# Autodesk Inventor assembly: yagi_Front
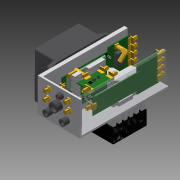
[picture p0: Inventor's stored thumbnail of the model, 180x180]
Saved by Autodesk Inventor 2014 (Build 180170000, 170)
## iProperties
Created: 2015-01-07
Part Number: yagi_Front
Document SubType Name: Assembly
Designer: Owner
Author: Owner
## Documents named in this file (22)
- C:\Users\Owner\Documents\APC\FrontEnd\IAM\Yagi\yagi_Front.iam
- C:\Users\Owner\Documents\APC\FrontEnd\IAM\Yagi\YagiBoard.iam
- C:\Users\Owner\Documents\APC\FrontEnd\IAM\Common\Yagi_BaseFrame.ipt
- C:\Users\Owner\Documents\APC\FrontEnd\IAM\Yagi\Yagi_Front_BackPlate.ipt
- C:\Users\Owner\Documents\APC\FrontEnd\IAM\Common\LED_Inset.ipt
- C:\Users\Owner\Documents\APC\FrontEnd\IAM\Common\BiglConnector.ipt
- C:\Users\Owner\Documents\APC\FrontEnd\IAM\Common\SmallConnector.ipt
- C:\Users\Owner\Documents\APC\FrontEnd\IAM\Yagi\SMA_Bulkhead.ipt
- C:\Users\Owner\Documents\APC\FrontEnd\IAM\Common\InjectorBoard2.iam
- C:\Users\Owner\Documents\APC\FrontEnd\IAM\Common\Peltier.ipt
- C:\Users\Owner\Documents\APC\FrontEnd\IAM\Common\PeltierPower.iam
- C:\Users\Owner\Documents\APC\FrontEnd\IAM\Common\Fan60.ipt
- C:\Users\Owner\Documents\APC\FrontEnd\IAM\Common\HeatSink60.ipt
- C:\Users\Owner\Documents\APC\FrontEnd\IAM\Common\NEAMBox.ipt
- C:\Users\Owner\Documents\APC\FrontEnd\IAM\Yagi\ColdFingerBase.ipt
- C:\Users\Owner\Documents\APC\FrontEnd\IAM\Yagi\ColdFingerStem.ipt
- C:\Users\Owner\Documents\APC\FrontEnd\IAM\Yagi\PeltierThermalSpacer.ipt
- C:\Users\Owner\Documents\APC\FrontEnd\IAM\Yagi\PeltierHeatSinkMount.ipt
- C:\Users\Owner\Documents\APC\FrontEnd\IAM\Yagi\YagiTop.ipt
- C:\Users\Owner\Documents\APC\FrontEnd\IAM\Common\PeltierController.iam
- C:\Users\Owner\Documents\APC\FrontEnd\IAM\Yagi\CavitySplitter.ipt
- C:\Users\Owner\Documents\APC\FrontEnd\IAM\Common\AmpPS.iam
## Components (27 placed, 21 different names)
1. YagiBoard:1 [sub-assembly] — Mate:47, Flush:16, Flush:17, Flush:48
2. Yagi_BaseFrame:1 — Flush:11, Mate:38, Flush:15, Mate:48, Flush:18, Flush:19, Flush:20, Flush:21, Mate:54, Flush:27, Flush:43, Flush:46, Mate:62
3. Yagi_BaseFrame:2 — Mate:47, Flush:16, Flush:17, Flush:20, Flush:21, Flush:22
4. Yagi_Front_BackPlate:1 — Mate:22, Mate:25, Mate:26, Mate:27, Mate:28, Mate:29, Mate:30, Mate:31, Flush:11, Mate:38, Flush:15, Mate:39, Mate:40, Mate:41, Mate:42, Mate:43, Mate:44, Mate:45, Mate:46, Angle:2, Angle:3, Angle:4, Angle:5, Flush:22, Flush:41, Flush:42
5. LED_Inset:2 — Mate:22, Mate:25
6. BiglConnector:1 — Mate:26, Mate:31
7. SmallConnector:1 — Mate:27, Mate:30
8. SmallConnector:2 — Mate:28, Mate:29
9. SMA_Bulkhead:1 — Mate:40, Mate:45, Angle:3
10. SMA_Bulkhead:2 — Mate:39, Mate:46, Angle:2
11. SMA_Bulkhead:3 — Mate:41, Mate:44, Angle:4
12. SMA_Bulkhead:4 — Mate:42, Mate:43, Angle:5
13. YagiBoard:2 [sub-assembly] — Mate:48, Flush:18, Flush:19
14. InjectorBoard2:1 [sub-assembly] — Mate:63, Flush:48, Mate:65, Flush:50
15. Peltier:1 — Flush:28, Flush:29, Flush:30, Flush:33, Flush:34, Flush:35
16. PeltierPower:1 [sub-assembly] — Mate:51, Mate:52, Mate:53
17. Fan60:1 — Mate:49, Flush:23, Flush:24, Flush:39, Flush:40, Flush:37, Flush:36
18. HeatSink60:1 — Mate:49, Flush:23, Flush:24, Mate:56, Flush:38
19. NEAMBox:1 — Mate:51, Mate:52, Mate:53, Mate:54, Flush:27, Mate:59, Mate:60, Flush:46
20. ColdFingerBase:1 — Flush:28, Flush:29, Flush:30, Mate:55, Flush:31, Mate:58
21. ColdFingerStem:1 — Mate:55, Flush:31, Mate:58
22. PeltierThermalSpacer:1 — Flush:33, Flush:34, Flush:35, Mate:56, Flush:36, Flush:37
23. PeltierHeatSinkMount:1 — Flush:38, Flush:39, Flush:40, Mate:57, Flush:44, Flush:45
24. YagiTop:1 — Flush:41, Flush:42, Flush:43, Mate:57, Flush:44, Flush:45, Mate:61, Flush:47
25. PeltierController:1 [sub-assembly] — Mate:59, Mate:60
26. CavitySplitter:1 — Mate:61, Mate:62, Mate:63, Flush:47, Mate:64, Flush:49, Flush:50
27. AmpPS:1 [sub-assembly] — Mate:64, Flush:49, Mate:65
## Relationships (73: Mate 35, Flush 34, Angle 4)
- Mate:22: Yagi_Front_BackPlate:1 ↔ LED_Inset:2
- Mate:25: Yagi_Front_BackPlate:1 ↔ LED_Inset:2
- Mate:26: Yagi_Front_BackPlate:1 ↔ BiglConnector:1
- Mate:27: Yagi_Front_BackPlate:1 ↔ SmallConnector:1
- Mate:28: Yagi_Front_BackPlate:1 ↔ SmallConnector:2
- Mate:29: Yagi_Front_BackPlate:1 ↔ SmallConnector:2
- Mate:30: Yagi_Front_BackPlate:1 ↔ SmallConnector:1
- Mate:31: Yagi_Front_BackPlate:1 ↔ BiglConnector:1
- Flush:11: Yagi_BaseFrame:1 ↔ Yagi_Front_BackPlate:1
- Mate:38: Yagi_BaseFrame:1 ↔ Yagi_Front_BackPlate:1
- Flush:15: Yagi_BaseFrame:1 ↔ Yagi_Front_BackPlate:1
- Mate:39: Yagi_Front_BackPlate:1 ↔ SMA_Bulkhead:2
- Mate:40: Yagi_Front_BackPlate:1 ↔ SMA_Bulkhead:1
- Mate:41: Yagi_Front_BackPlate:1 ↔ SMA_Bulkhead:3
- Mate:42: Yagi_Front_BackPlate:1 ↔ SMA_Bulkhead:4
- Mate:43: Yagi_Front_BackPlate:1 ↔ SMA_Bulkhead:4
- Mate:44: Yagi_Front_BackPlate:1 ↔ SMA_Bulkhead:3
- Mate:45: Yagi_Front_BackPlate:1 ↔ SMA_Bulkhead:1
- Mate:46: Yagi_Front_BackPlate:1 ↔ SMA_Bulkhead:2
- Angle:2 (0 deg): Yagi_Front_BackPlate:1 ↔ SMA_Bulkhead:2
- Angle:3 (0 deg): Yagi_Front_BackPlate:1 ↔ SMA_Bulkhead:1
- Angle:4 (0 deg): Yagi_Front_BackPlate:1 ↔ SMA_Bulkhead:3
- Angle:5 (0 deg): Yagi_Front_BackPlate:1 ↔ SMA_Bulkhead:4
- Mate:47 (3.175 mm): YagiBoard:1 ↔ Yagi_BaseFrame:2
- Flush:16: YagiBoard:1 ↔ Yagi_BaseFrame:2
- Flush:17 (3.175 mm): YagiBoard:1 ↔ Yagi_BaseFrame:2
- Mate:48 (3.175 mm): Yagi_BaseFrame:1 ↔ YagiBoard:2
- Flush:18 (3.175 mm): Yagi_BaseFrame:1 ↔ YagiBoard:2
- Flush:19: Yagi_BaseFrame:1 ↔ YagiBoard:2
- Flush:20: Yagi_BaseFrame:1 ↔ Yagi_BaseFrame:2
- Flush:21: Yagi_BaseFrame:1 ↔ Yagi_BaseFrame:2
- Flush:22: Yagi_BaseFrame:2 ↔ Yagi_Front_BackPlate:1
- Mate:49: Fan60:1 ↔ HeatSink60:1
- Flush:23 (-1 mm): Fan60:1 ↔ HeatSink60:1
- Flush:24 (-2 mm): Fan60:1 ↔ HeatSink60:1
- Mate:51: PeltierPower:1 ↔ NEAMBox:1
- Mate:52 (6.35 mm): PeltierPower:1 ↔ NEAMBox:1
- Mate:53 (3.175 mm): PeltierPower:1 ↔ NEAMBox:1
- Mate:54: Yagi_BaseFrame:1 ↔ NEAMBox:1
- Flush:27 (-3.175 mm): Yagi_BaseFrame:1 ↔ NEAMBox:1
- Flush:28: Peltier:1 ↔ ColdFingerBase:1
- Flush:29: Peltier:1 ↔ ColdFingerBase:1
- Flush:30: Peltier:1 ↔ ColdFingerBase:1
- Mate:55: ColdFingerBase:1 ↔ ColdFingerStem:1
- Flush:31: ColdFingerBase:1 ↔ ColdFingerStem:1
- Mate:58: ColdFingerBase:1 ↔ ColdFingerStem:1
- Flush:33: Peltier:1 ↔ PeltierThermalSpacer:1
- Flush:34: Peltier:1 ↔ PeltierThermalSpacer:1
- Flush:35: Peltier:1 ↔ PeltierThermalSpacer:1
- Mate:56: HeatSink60:1 ↔ PeltierThermalSpacer:1
- Flush:36 (10 mm): Fan60:1 ↔ PeltierThermalSpacer:1
- Flush:37 (10 mm): Fan60:1 ↔ PeltierThermalSpacer:1
- Flush:38: HeatSink60:1 ↔ PeltierHeatSinkMount:1
- Flush:39: Fan60:1 ↔ PeltierHeatSinkMount:1
- Flush:40: Fan60:1 ↔ PeltierHeatSinkMount:1
- Flush:41: Yagi_Front_BackPlate:1 ↔ YagiTop:1
- Flush:42: Yagi_Front_BackPlate:1 ↔ YagiTop:1
- Flush:43: Yagi_BaseFrame:1 ↔ YagiTop:1
- Mate:57: PeltierHeatSinkMount:1 ↔ YagiTop:1
- Flush:44: PeltierHeatSinkMount:1 ↔ YagiTop:1
- Flush:45: PeltierHeatSinkMount:1 ↔ YagiTop:1
- Mate:59: NEAMBox:1 ↔ PeltierController:1
- Mate:60 (6.35 mm): NEAMBox:1 ↔ PeltierController:1
- Flush:46 (38.1 mm): Yagi_BaseFrame:1 ↔ NEAMBox:1
- Mate:61: YagiTop:1 ↔ CavitySplitter:1
- Mate:62 (22.86 mm): Yagi_BaseFrame:1 ↔ CavitySplitter:1
- Mate:63: InjectorBoard2:1 ↔ CavitySplitter:1
- Flush:47: YagiTop:1 ↔ CavitySplitter:1
- Flush:48: YagiBoard:1 ↔ InjectorBoard2:1
- Mate:64 (1.5875 mm): CavitySplitter:1 ↔ AmpPS:1
- Flush:49: CavitySplitter:1 ↔ AmpPS:1
- Mate:65 (1.5875 mm): InjectorBoard2:1 ↔ AmpPS:1
- Flush:50 (3.175 mm): InjectorBoard2:1 ↔ CavitySplitter:1
